# Autodesk Inventor assembly: Assembly2
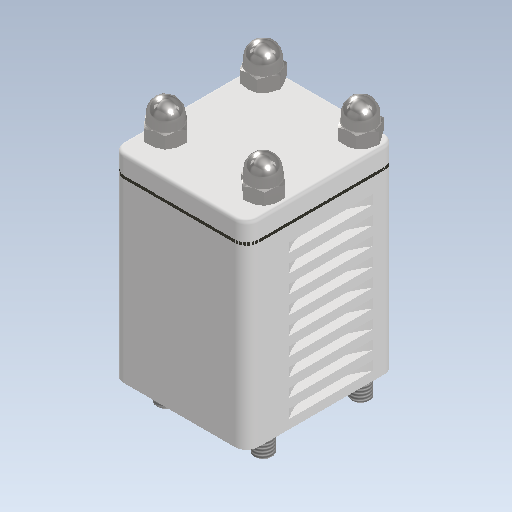
[picture p0: Inventor's stored thumbnail of the model, 512x512]
Saved by Autodesk Inventor 2020 (Build 240168000, 168)
## iProperties
Created: 2020-08-14
Part Number: Assembly2
Document SubType Name: Assembly
Designer: benny
Author: benny
## Documents named in this file (6)
- C:\Users\benny\Desktop\importantmajorprojecthev_june\engine\assembly\BENNY S L_JUNE BATCH_Assembly2.iam
- C:\Users\benny\Desktop\importantmajorprojecthev_june\engine\others\Benny S L_JUNE BATCH_ cylinder\Benny S L_JUNE BATCH_cylinder head gasket.ipt
- C:\Users\benny\Desktop\importantmajorprojecthev_june\engine\others\Benny S L_JUNE BATCH_ cylinder\Benny S L_JUNE BATCH_cylinder head.ipt
- C:\Users\benny\Desktop\importantmajorprojecthev_june\engine\others\Benny S L_JUNE BATCH_ cylinder\Benny S L_JUNE BATCH_cylinder.ipt
- C:\Users\benny\Desktop\importantmajorprojecthev_june\engine\others\Benny S L_JUNE BATCH_ cylinder\Benny S L_JUNE BATCH_cylinder head bolt.ipt
- C:\Users\benny\Documents\Inventor\Content Center Files\R2020\en-US\DIN 1587\DIN 1587 - M6 x 1.ipt
## Components (11 placed, 5 different names)
1. Benny S L_JUNE BATCH_cylinder head gasket:1 — Mate:1, Mate:2, Mate:3, Mate:6
2. Benny S L_JUNE BATCH_cylinder head:1 — Mate:4, Mate:5, Mate:6, Mate:7, Mate:11, Mate:20, Mate:21, Mate:22, Mate:23, Mate:24
3. Benny S L_JUNE BATCH_cylinder:1 — Mate:1, Mate:2, Mate:3, Mate:4, Mate:5, Mate:19
4. Benny S L_JUNE BATCH_cylinder head bolt:1 — Mate:7, Mate:8, Mate:9, Mate:10
5. Benny S L_JUNE BATCH_cylinder head bolt:2 — Mate:12, Mate:13, Mate:14, Mate:23
6. Benny S L_JUNE BATCH_cylinder head bolt:3 — Mate:15, Mate:16, Mate:21
7. Benny S L_JUNE BATCH_cylinder head bolt:4 — Mate:17, Mate:18, Mate:19
8. DIN 1587 M6:1 — Mate:8, Mate:9, Mate:10, Mate:11
9. DIN 1587 M6:2 — Mate:12, Mate:13, Mate:14, Mate:24
10. DIN 1587 M6:3 — Mate:17, Mate:18, Mate:20
11. DIN 1587 M6:4 — Mate:15, Mate:16, Mate:22
## Relationships (24: Mate 24)
- Mate:1: Benny S L_JUNE BATCH_cylinder head gasket:1 ↔ Benny S L_JUNE BATCH_cylinder:1
- Mate:2: Benny S L_JUNE BATCH_cylinder head gasket:1 ↔ Benny S L_JUNE BATCH_cylinder:1
- Mate:3: Benny S L_JUNE BATCH_cylinder head gasket:1 ↔ Benny S L_JUNE BATCH_cylinder:1
- Mate:4: Benny S L_JUNE BATCH_cylinder head:1 ↔ Benny S L_JUNE BATCH_cylinder:1
- Mate:5: Benny S L_JUNE BATCH_cylinder head:1 ↔ Benny S L_JUNE BATCH_cylinder:1
- Mate:6: Benny S L_JUNE BATCH_cylinder head gasket:1 ↔ Benny S L_JUNE BATCH_cylinder head:1
- Mate:7: Benny S L_JUNE BATCH_cylinder head:1 ↔ Benny S L_JUNE BATCH_cylinder head bolt:1
- Mate:8: Benny S L_JUNE BATCH_cylinder head bolt:1 ↔ DIN 1587 M6:1
- Mate:9: Benny S L_JUNE BATCH_cylinder head bolt:1 ↔ DIN 1587 M6:1
- Mate:10: Benny S L_JUNE BATCH_cylinder head bolt:1 ↔ DIN 1587 M6:1
- Mate:11: Benny S L_JUNE BATCH_cylinder head:1 ↔ DIN 1587 M6:1
- Mate:12: Benny S L_JUNE BATCH_cylinder head bolt:2 ↔ DIN 1587 M6:2
- Mate:13: Benny S L_JUNE BATCH_cylinder head bolt:2 ↔ DIN 1587 M6:2
- Mate:14: Benny S L_JUNE BATCH_cylinder head bolt:2 ↔ DIN 1587 M6:2
- Mate:15: Benny S L_JUNE BATCH_cylinder head bolt:3 ↔ DIN 1587 M6:4
- Mate:16: Benny S L_JUNE BATCH_cylinder head bolt:3 ↔ DIN 1587 M6:4
- Mate:17: Benny S L_JUNE BATCH_cylinder head bolt:4 ↔ DIN 1587 M6:3
- Mate:18: Benny S L_JUNE BATCH_cylinder head bolt:4 ↔ DIN 1587 M6:3
- Mate:19: Benny S L_JUNE BATCH_cylinder:1 ↔ Benny S L_JUNE BATCH_cylinder head bolt:4
- Mate:20: Benny S L_JUNE BATCH_cylinder head:1 ↔ DIN 1587 M6:3
- Mate:21: Benny S L_JUNE BATCH_cylinder head:1 ↔ Benny S L_JUNE BATCH_cylinder head bolt:3
- Mate:22: Benny S L_JUNE BATCH_cylinder head:1 ↔ DIN 1587 M6:4
- Mate:23: Benny S L_JUNE BATCH_cylinder head:1 ↔ Benny S L_JUNE BATCH_cylinder head bolt:2
- Mate:24: Benny S L_JUNE BATCH_cylinder head:1 ↔ DIN 1587 M6:2
